# Autodesk Inventor assembly: Stand
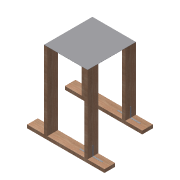
[picture p0: Inventor's stored thumbnail of the model, 180x180]
Saved by Autodesk Inventor 2017 (Build 210142000, 142)
## iProperties
Created: 2017-05-22
Part Number: Stand
Document SubType Name: Assembly
Designer: krosie
Author: krosie
## Documents named in this file (7)
- C:\Users\krosie\Google Drive\HERA\hera-cad\Node\Fan\Mount\Stand.iam
- FrontStand.iam
- C:\Users\krosie\Google Drive\HERA\hera-cad\Node\Fan\Mount\BaseStand.ipt
- C:\Users\krosie\Google Drive\HERA\hera-cad\Node\Fan\Mount\UprightStand_Back.ipt
- C:\Users\krosie\Google Drive\HERA\hera-cad\Node\Fan\Mount\UprightStand_Front.ipt
- C:\Users\krosie\Google Drive\HERA\hera-cad\Node\Fan\Mount\StandPlatform.ipt
- C:\Users\krosie\Google Drive\HERA\hera-cad\Node\Fan\Mount\80mmCornerBracket.ipt
## Components (11 placed, 5 different names)
1. BaseStand:1 — Mate:1, Flush:1, Flush:2, Mate:2, Mate:3, Flush:3, Flush:4, Flush:5, Mate:7, Mate:9, Flush:12, Flush:13
2. BaseStand:2 — Mate:1, Flush:1, Flush:2, Mate:5, Mate:6, Flush:8, Flush:9, Mate:11, Mate:13, Flush:10, Flush:11
3. UprightStand_Back:1 — Mate:2, Flush:3, Mate:4, Flush:5, Flush:6
4. UprightStand_Back:2 — Mate:3, Flush:4, Mate:4, Flush:7, Mate:8, Mate:10
5. UprightStand_Front:1 — Flush:6, Mate:5, Flush:8
6. UprightStand_Front:2 — Flush:7, Mate:6, Flush:9, Mate:12, Mate:14
7. StandPlatform:1
8. 30mmCornerBracket:1 — Mate:9, Mate:10, Flush:12
9. 30mmCornerBracket:2 — Mate:11, Mate:12, Flush:11
10. 30mmCornerBracket:3 — Mate:13, Mate:14, Flush:10
11. 30mmCornerBracket:4 — Mate:7, Mate:8, Flush:13
## Relationships (27: Mate 14, Flush 13)
- Mate:1 (-500 mm): BaseStand:1 ↔ BaseStand:2
- Flush:1: BaseStand:1 ↔ BaseStand:2
- Flush:2 (150 mm): BaseStand:1 ↔ BaseStand:2
- Mate:2: BaseStand:1 ↔ UprightStand_Back:1
- Mate:3: BaseStand:1 ↔ UprightStand_Back:2
- Flush:3: BaseStand:1 ↔ UprightStand_Back:1
- Flush:4: BaseStand:1 ↔ UprightStand_Back:2
- Mate:4 (-450 mm): UprightStand_Back:1 ↔ UprightStand_Back:2
- Flush:5 (-175 mm): BaseStand:1 ↔ UprightStand_Back:1
- Flush:6: UprightStand_Back:1 ↔ UprightStand_Front:1
- Flush:7: UprightStand_Back:2 ↔ UprightStand_Front:2
- Mate:5: BaseStand:2 ↔ UprightStand_Front:1
- Mate:6: BaseStand:2 ↔ UprightStand_Front:2
- Flush:8: BaseStand:2 ↔ UprightStand_Front:1
- Flush:9: BaseStand:2 ↔ UprightStand_Front:2
- Mate:7: BaseStand:1 ↔ 30mmCornerBracket:4
- Mate:8: UprightStand_Back:2 ↔ 30mmCornerBracket:4
- Mate:9: BaseStand:1 ↔ 30mmCornerBracket:1
- Mate:10: UprightStand_Back:2 ↔ 30mmCornerBracket:1
- Mate:11: BaseStand:2 ↔ 30mmCornerBracket:2
- Mate:12: UprightStand_Front:2 ↔ 30mmCornerBracket:2
- Mate:13: BaseStand:2 ↔ 30mmCornerBracket:3
- Mate:14: UprightStand_Front:2 ↔ 30mmCornerBracket:3
- Flush:10 (47.5 mm): BaseStand:2 ↔ 30mmCornerBracket:3
- Flush:11 (47.5 mm): BaseStand:2 ↔ 30mmCornerBracket:2
- Flush:12 (47.5 mm): BaseStand:1 ↔ 30mmCornerBracket:1
- Flush:13 (47.5 mm): BaseStand:1 ↔ 30mmCornerBracket:4
